# Autodesk Inventor assembly: CAM1
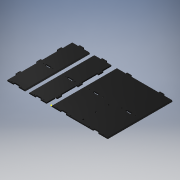
[picture p0: Inventor's stored thumbnail of the model, 180x180]
Saved by Autodesk Inventor 2017 (Build 210142000, 142)
## iProperties
Created: 2019-05-25
Part Number: CAM1
Document SubType Name: Assembly
Designer: 3D Printer
Author: 3D Printer
## Documents named in this file (4)
- C:\Users\3D Printer\Documents\GitHub\tr2\Body 2.0\CAM1.iam
- C:\Users\3D Printer\Documents\GitHub\tr2\Body 2.0\BA05.ipt
- C:\Users\3D Printer\Documents\GitHub\tr2\Body 2.0\BA06.ipt
- C:\Users\3D Printer\Documents\GitHub\tr2\Body 2.0\BA03.ipt
## Components (3 placed, 3 different names)
1. BA05:1 — Mate:3, Mate:13, Mate:14, Mate:15, Flush:3
2. BA06:1 — Mate:1, Flush:2, Mate:12, Mate:15, Flush:3
3. BA03:1 — Mate:5, Flush:2, Mate:12
## Relationships (9: Mate 7, Flush 2)
- Mate:1: BA06:1
- Mate:3: BA05:1
- Mate:5: BA03:1
- Flush:2: BA06:1 ↔ BA03:1
- Mate:12 (20 mm): BA06:1 ↔ BA03:1
- Mate:13: BA05:1
- Mate:14: BA05:1
- Mate:15 (20 mm): BA05:1 ↔ BA06:1
- Flush:3: BA05:1 ↔ BA06:1
